# Autodesk Inventor assembly: Y_rail_Assembly_Rev3
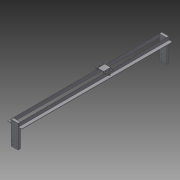
[picture p0: Inventor's stored thumbnail of the model, 180x180]
Saved by Autodesk Inventor 2015 (Build 190159000, 159)
## iProperties
Created: 2017-01-11
Part Number: Y_rail_Assembly_Rev3
Document SubType Name: Assembly
Designer: Guy
Author: Guy
## Documents named in this file (6)
- C:\Users\Guy\Documents\Fourth Year\Capstone\git\Capstone-Project\doc\CAD\LowLevel_Rev3\Y_rail_Assembly_Rev3.iam
- C:\Users\Guy\Documents\Fourth Year\Capstone\git\Capstone-Project\doc\CAD\LowLevel_Rev3\Y_Rail-SquareBar-Rev3.ipt
- C:\Users\Guy\Documents\Fourth Year\Capstone\git\Capstone-Project\doc\CAD\LowLevel_Rev3\Arm-SquareBar-Rev3.ipt
- C:\Users\Guy\Documents\Fourth Year\Capstone\git\Capstone-Project\doc\CAD\LowLevel_Rev3\XY_Wheel-SquareBar-Rev3.ipt
- C:\Users\Guy\Documents\Fourth Year\Capstone\git\Capstone-Project\doc\CAD\LowLevel_Rev3\EE_Base-SquareBar-Rev3.ipt
- C:\Users\Guy\Documents\Fourth Year\Capstone\git\Capstone-Project\doc\CAD\LowLevel_Rev3\Y_Rail_Alignement _Connector_SquareBar-Rev3.ipt
## Components (13 placed, 5 different names)
1. Y_Rail-SquareBar-Rev3:1 — Mate:2, Mate:5, Mate:6, Tangent:1, Tangent:2, Mate:11, Tangent:6
2. Y_Rail-SquareBar-Rev3:2 — Mate:1, Mate:4, Mate:7, Mate:8, Tangent:3, Tangent:4, Mate:12, Tangent:5
3. Arm-SquareBar-Rev3:1 — Mate:1, Mate:2, Mate:5, Flush:1, Mate:7
4. Arm-SquareBar-Rev3:2 — Mate:4, Mate:6, Flush:1, Mate:8
5. XY_Wheel-SquareBar-Rev3:1 — Tangent:1, Mate:9, Flush:2, Mate:14, Mate:15, Mate:20
6. XY_Wheel-SquareBar-Rev3:2 — Tangent:4, Mate:9, Flush:4, Mate:17
7. XY_Wheel-SquareBar-Rev3:3 — Tangent:3, Mate:10, Mate:12, Flush:4, Mate:18
8. XY_Wheel-SquareBar-Rev3:4 — Tangent:2, Mate:10, Mate:11, Flush:2, Mate:13, Mate:21
9. EE_Base-SquareBar-Rev3:1 — Mate:13, Mate:14, Mate:15
10. XY_Wheel-SquareBar-Rev3:5 — Tangent:5, Mate:16, Mate:23
11. Y_Rail_Alignement _Connector_SquareBar-Rev3:1 — Mate:16, Mate:17, Mate:18, Mate:23
12. XY_Wheel-SquareBar-Rev3:6 — Tangent:6, Mate:19, Mate:22
13. Y_Rail_Alignement _Connector_SquareBar-Rev3:2 — Mate:19, Mate:20, Mate:21, Mate:22
## Relationships (31: Mate 22, Tangent 6, Flush 3)
- Mate:1: Y_Rail-SquareBar-Rev3:2 ↔ Arm-SquareBar-Rev3:1
- Mate:2: Y_Rail-SquareBar-Rev3:1 ↔ Arm-SquareBar-Rev3:1
- Mate:4: Y_Rail-SquareBar-Rev3:2 ↔ Arm-SquareBar-Rev3:2
- Mate:5: Y_Rail-SquareBar-Rev3:1 ↔ Arm-SquareBar-Rev3:1
- Mate:6: Y_Rail-SquareBar-Rev3:1 ↔ Arm-SquareBar-Rev3:2
- Flush:1: Arm-SquareBar-Rev3:1 ↔ Arm-SquareBar-Rev3:2
- Mate:7: Y_Rail-SquareBar-Rev3:2 ↔ Arm-SquareBar-Rev3:1
- Mate:8: Y_Rail-SquareBar-Rev3:2 ↔ Arm-SquareBar-Rev3:2
- Tangent:1: Y_Rail-SquareBar-Rev3:1 ↔ XY_Wheel-SquareBar-Rev3:1
- Tangent:2: Y_Rail-SquareBar-Rev3:1 ↔ XY_Wheel-SquareBar-Rev3:4
- Tangent:3: Y_Rail-SquareBar-Rev3:2 ↔ XY_Wheel-SquareBar-Rev3:3
- Tangent:4: Y_Rail-SquareBar-Rev3:2 ↔ XY_Wheel-SquareBar-Rev3:2
- Mate:9: XY_Wheel-SquareBar-Rev3:1 ↔ XY_Wheel-SquareBar-Rev3:2
- Mate:10: XY_Wheel-SquareBar-Rev3:3 ↔ XY_Wheel-SquareBar-Rev3:4
- Mate:11 (1.75 mm): Y_Rail-SquareBar-Rev3:1 ↔ XY_Wheel-SquareBar-Rev3:4
- Flush:2: XY_Wheel-SquareBar-Rev3:1 ↔ XY_Wheel-SquareBar-Rev3:4
- Mate:12 (1.75 mm): Y_Rail-SquareBar-Rev3:2 ↔ XY_Wheel-SquareBar-Rev3:3
- Flush:4: XY_Wheel-SquareBar-Rev3:2 ↔ XY_Wheel-SquareBar-Rev3:3
- Mate:13: XY_Wheel-SquareBar-Rev3:4 ↔ EE_Base-SquareBar-Rev3:1
- Mate:14: XY_Wheel-SquareBar-Rev3:1 ↔ EE_Base-SquareBar-Rev3:1
- Mate:15 (2.25 mm): XY_Wheel-SquareBar-Rev3:1 ↔ EE_Base-SquareBar-Rev3:1
- Tangent:5: Y_Rail-SquareBar-Rev3:2 ↔ XY_Wheel-SquareBar-Rev3:5
- Mate:16: XY_Wheel-SquareBar-Rev3:5 ↔ Y_Rail_Alignement _Connector_SquareBar-Rev3:1
- Mate:17: XY_Wheel-SquareBar-Rev3:2 ↔ Y_Rail_Alignement _Connector_SquareBar-Rev3:1
- Mate:18: XY_Wheel-SquareBar-Rev3:3 ↔ Y_Rail_Alignement _Connector_SquareBar-Rev3:1
- Tangent:6: Y_Rail-SquareBar-Rev3:1 ↔ XY_Wheel-SquareBar-Rev3:6
- Mate:19: XY_Wheel-SquareBar-Rev3:6 ↔ Y_Rail_Alignement _Connector_SquareBar-Rev3:2
- Mate:20: XY_Wheel-SquareBar-Rev3:1 ↔ Y_Rail_Alignement _Connector_SquareBar-Rev3:2
- Mate:21: XY_Wheel-SquareBar-Rev3:4 ↔ Y_Rail_Alignement _Connector_SquareBar-Rev3:2
- Mate:22 (10 mm): XY_Wheel-SquareBar-Rev3:6 ↔ Y_Rail_Alignement _Connector_SquareBar-Rev3:2
- Mate:23 (10 mm): XY_Wheel-SquareBar-Rev3:5 ↔ Y_Rail_Alignement _Connector_SquareBar-Rev3:1
